# Autodesk Inventor assembly: Wheel
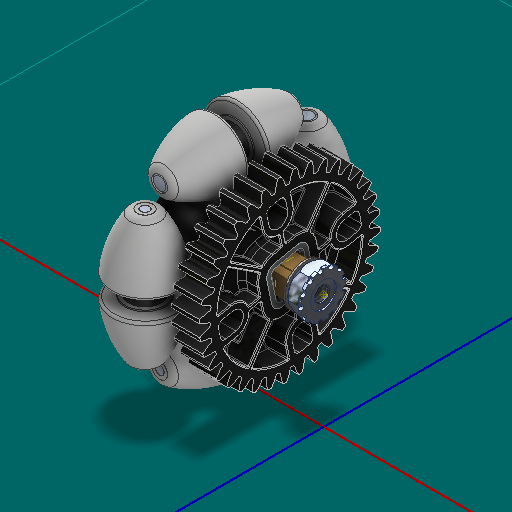
[picture p0: Inventor's stored thumbnail of the model, 512x512]
Saved by Autodesk Inventor 2025 (Build 290162000, 162)
## iProperties
Created: 2024-10-18
Part Number: Wheel
Document SubType Name: Assembly
Designer: averey
Author: averey
## Documents named in this file (7)
- C:\Users\avere\VEX\High Stakes\CAD\V2\Chassis\Drivebay Left\Wheel.iam
- C:\Users\avere\VEX\High Stakes\CAD\ROBOPROS-CAD-Inventor\Modified Parts\Half Cut HS 36T Gear, No Insert.ipt
- C:\Users\avere\VEX\High Stakes\CAD\ROBOPROS-CAD-Inventor\Motion\HS Shaft Adapter Circle.ipt
- C:\Users\avere\VEX\High Stakes\CAD\ROBOPROS-CAD-Inventor\Structure\Hardware\Nut Keps.ipt
- C:\Users\avere\VEX\High Stakes\CAD\ROBOPROS-CAD-Inventor\Motion\Spacers\Washer Steel\SWasher .375 OD x .015625.ipt
- C:\Users\avere\vex_robotics_high_stakes\hardware\cad\robpros_cad_lib\Motion\Spacers\Washer Steel.ipt
- C:\Users\avere\VEX\High Stakes\CAD\ROBOPROS-CAD-Inventor\Motion\Wheels\Omni Wheel\2.00 Omni AS, No Insert.ipt
## Components (7 placed, 5 different names)
1. Half Cut HS 36T Gear, No Insert:1
2. HS Shaft Adapter Circle:1
3. Nut Keps:1 — Mate:1
4. SWasher .375 OD x .015625:1
5. 2.00 Omni AS, No Insert:1
6. SWasher .375 OD x .015625:2
7. HS Shaft Adapter Circle:2
## Relationships (8: Insert 6, Angle 1, Mate 1)
- [Angle] (0 deg): Half Cut HS 36T Gear, No Insert:1 ↔ HS Shaft Adapter Circle:1
- [Insert]: HS Shaft Adapter Circle:1 ↔ HS Shaft Adapter Circle:2
- [Insert]: Nut Keps:1 ↔ SWasher .375 OD x .015625:2
- [Insert]: SWasher .375 OD x .015625:2 ↔ HS Shaft Adapter Circle:2
- [Insert]: HS Shaft Adapter Circle:1 ↔ SWasher .375 OD x .015625:1
- [Insert]: SWasher .375 OD x .015625:1 ↔ 2.00 Omni AS, No Insert:1
- [Insert]: Half Cut HS 36T Gear, No Insert:1 ↔ 2.00 Omni AS, No Insert:1
- Mate:1: Nut Keps:1
